# Autodesk Inventor assembly: xx
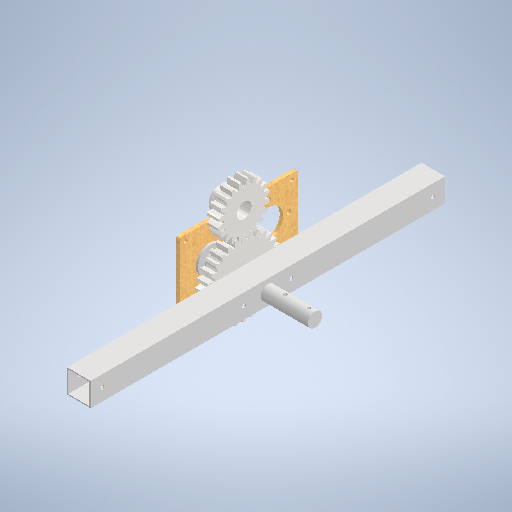
[picture p0: Inventor's stored thumbnail of the model, 512x512]
Saved by Autodesk Inventor 2025.1 (Build 291241000, 241)
## iProperties
Created: 2024-12-04
Part Number: xx
Document SubType Name: Assembly
Designer: yuki0520
Author: yuki0520
## Documents named in this file (6)
- C:\Users\yuki0520\OneDrive\ドキュメント\Inventor\2025_nhk\tanaka\nageru\pakuriz\xx.iam
- C:\Users\yuki0520\OneDrive\ドキュメント\Inventor\2025_nhk\tanaka\nageru\pakuriz\xx_jiku_kakudo.ipt
- C:\Users\yuki0520\OneDrive\ドキュメント\Inventor\2025_nhk\tanaka\nageru\pakuriz\xx_shita.ipt
- C:\Users\yuki0520\OneDrive\ドキュメント\Inventor\2025_nhk\tanaka\nageru\pakuriz\xx_gear.iam
- C:\Users\yuki0520\OneDrive\ドキュメント\Inventor\2025_nhk\tanaka\nageru\pakuriz\xx_plate_motor.ipt
- C:\Users\yuki0520\OneDrive\ドキュメント\Inventor\2025_nhk\tanaka\nageru\pakuriz\bear_12_18.ipt
## Components (5 placed, 5 different names)
1. xx_jiku_kakudo:1 — メイト:1, メイト:2, メイト:3, メイト:7
2. xx_shita:1 — メイト:2, 挿入:1
3. xx_gear:1 [sub-assembly] — メイト:1, メイト:3, 挿入:1
4. xx_plate_motor:1 — メイト:5, メイト:6
5. bear_12_18:1 — メイト:5, メイト:6, メイト:7
## Relationships (7: Mate 6, Insert 1)
- メイト:1 [Mate]: xx_jiku_kakudo:1 ↔ xx_gear:1
- メイト:2 [Mate]: xx_jiku_kakudo:1 ↔ xx_shita:1
- メイト:3 [Mate]: xx_jiku_kakudo:1 ↔ xx_gear:1
- メイト:5 [Mate]: xx_plate_motor:1 ↔ bear_12_18:1
- メイト:6 [Mate]: xx_plate_motor:1 ↔ bear_12_18:1
- メイト:7 [Mate]: xx_jiku_kakudo:1 ↔ bear_12_18:1
- 挿入:1 [Insert]: xx_shita:1 ↔ xx_gear:1
